# Autodesk Inventor assembly: A2017_T5_04
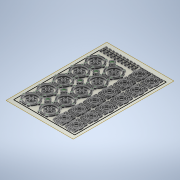
[picture p0: Inventor's stored thumbnail of the model, 180x180]
Saved by Autodesk Inventor 2022.3 (Build 263350000, 350)
## iProperties
Created: 2022-09-28
Part Number: A2017_T5_04
Document SubType Name: Assembly
Designer: Masato
Author: Masato
## Documents named in this file (7)
- C:\Users\Masato\Documents\Inventor\CIT Brains\SUSTAINA-OP - mod\Cam\A2017_T5\A2017_T5_04.iam
- C:\Users\Masato\Documents\Inventor\CIT Brains\SUSTAINA-OP - mod\Cam\DisposableBoard.ipt
- C:\Users\Masato\Documents\Inventor\CIT Brains\SUSTAINA-OP - mod\UpperBody\Trunk\CrossRollerBearing\Inner_support_stand.ipt
- C:\Users\Masato\Documents\Inventor\CIT Brains\SUSTAINA-OP - mod\UpperBody\Trunk\CrossRollerBearing\Outer_support_stand.ipt
- C:\Users\Masato\Documents\Inventor\CIT Brains\SUSTAINA-OP - mod\UpperBody\UpperBody_horn_frame.ipt
- C:\Users\Masato\Documents\Inventor\CIT Brains\SUSTAINA-OP - mod\LowerBody\Foot\Foot_root_block.ipt
- C:\Users\Masato\Documents\Inventor\CIT Brains\SUSTAINA-OP - mod\LowerBody\Knee\Knee_clamp.ipt
## Components (48 placed, 6 different names)
1. DisposableBoard:1 — フラッシュ:1, フラッシュ:2, フラッシュ:3, フラッシュ:4, Tangent:1, Tangent:2, Tangent:3, Flush:5, Flush:6, Mate:6, Mate:7, Flush:7
2. Inner_support_stand:1 — Mate:2, Insert:1
3. Outer_support_stand:1 — Mate:1, Insert:1, Tangent:1, Tangent:2, Tangent:3
4. Inner_support_stand:2
5. Outer_support_stand:2 — Tangent:4
6. Inner_support_stand:3
7. Outer_support_stand:3
8. Inner_support_stand:4
9. Outer_support_stand:4
10. Inner_support_stand:5
11. Outer_support_stand:5
12. Inner_support_stand:6
13. Outer_support_stand:6
14. Inner_support_stand:7
15. Outer_support_stand:7
16. Inner_support_stand:8
17. Outer_support_stand:8
18. Inner_support_stand:9
19. Outer_support_stand:9
20. Inner_support_stand:10
21. Outer_support_stand:10
22. UpperBody_horn_frame:1 — Mate:3, Flush:5, Tangent:4
23. UpperBody_horn_frame:2
24. UpperBody_horn_frame:3
25. UpperBody_horn_frame:4
26. UpperBody_horn_frame:5
27. UpperBody_horn_frame:6
28. UpperBody_horn_frame:7
29. UpperBody_horn_frame:8
30. UpperBody_horn_frame:9
31. UpperBody_horn_frame:10
32. UpperBody_horn_frame:11
33. UpperBody_horn_frame:12
34. Knee_clamp:1 — Mate:4, Mate:6, Mate:7
35. Knee_clamp:2
36. Knee_clamp:3
37. Knee_clamp:4
38. Knee_clamp:5
39. Foot_root_block:1 — Mate:5, Flush:6, Flush:7
40. Foot_root_block:2
41. Foot_root_block:3
42. Foot_root_block:4
43. Foot_root_block:5
44. Foot_root_block:6
45. Foot_root_block:7
46. Foot_root_block:8
47. Foot_root_block:9
48. Foot_root_block:10
## Component patterns: (10 elements, first: Inner_support_stand:1 + Outer_support_stand:1), (12 elements, first: UpperBody_horn_frame:1), (5 elements, first: Knee_clamp:1), (10 elements, first: Foot_root_block:1)
## Relationships (19: Flush 7, Mate 7, Tangent 4, Insert 1)
- フラッシュ:1 [Flush]: DisposableBoard:1
- フラッシュ:2 [Flush]: DisposableBoard:1
- フラッシュ:3 [Flush]: DisposableBoard:1
- フラッシュ:4 [Flush]: DisposableBoard:1
- Mate:1: Outer_support_stand:1
- Mate:2: Inner_support_stand:1
- Insert:1: Inner_support_stand:1 ↔ Outer_support_stand:1
- Mate:3: UpperBody_horn_frame:1
- Tangent:1 (2 mm): DisposableBoard:1 ↔ Outer_support_stand:1
- Tangent:2 (2 mm): DisposableBoard:1 ↔ Outer_support_stand:1
- Tangent:3 (2 mm): DisposableBoard:1 ↔ Outer_support_stand:1
- Flush:5 (-2 mm): DisposableBoard:1 ↔ UpperBody_horn_frame:1
- Tangent:4 (2.1 mm): Outer_support_stand:2 ↔ UpperBody_horn_frame:1
- Mate:4: Knee_clamp:1
- Mate:5: Foot_root_block:1
- Flush:6 (2 mm): DisposableBoard:1 ↔ Foot_root_block:1
- Mate:6 (-51.568 mm): DisposableBoard:1 ↔ Knee_clamp:1
- Mate:7 (-60.5 mm): DisposableBoard:1 ↔ Knee_clamp:1
- Flush:7 (2 mm): DisposableBoard:1 ↔ Foot_root_block:1
